# Autodesk Inventor assembly: ProvedoSenzor
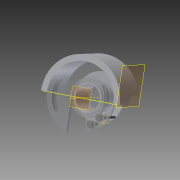
[picture p0: Inventor's stored thumbnail of the model, 180x180]
Saved by Autodesk Inventor 2015 (Build 190159000, 159)
## iProperties
Created: 2014-11-14
Part Number: ProvedoSenzor
Document SubType Name: Assembly
Designer: laca
Author: laca
## Documents named in this file (12)
- C:\Users\laca\Desktop\iRoobo2014Ver3\ProvedoSenzor.iam
- C:\Users\laca\Desktop\iRoobo2014Ver3\BurkolatPVCszenzor.ipt
- C:\Users\laca\Desktop\iRoobo2014Ver3\PorvedoRogzitesAVazhoz.ipt
- C:\Users\laca\Desktop\iRoobo2014Ver3\BurkolatPVCszenzorFedel.ipt
- C:\Users\laca\Desktop\iRoobo2014Ver3\SzenzorSzuportKerek.ipt
- C:\Users\laca\Desktop\iRoobo2014Ver3\InkrementalisOptikaiErzekelo.ipt
- C:\Users\laca\Desktop\iRoobo2014Ver3\InkrementalisFolia.ipt
- C:\Users\laca\Desktop\iRoobo2014Ver3\MerevitesInkrementalisFolia.ipt
- C:\Users\laca\Desktop\iRoobo2014Ver3\Alatet3csavarhoz.ipt
- C:\Users\laca\Desktop\iRoobo2014Ver3\Fi3es40mmcsavar Hexagon.ipt
- C:\Users\laca\Desktop\iRoobo2014Ver3\3asAnya.ipt
- C:\Users\laca\Desktop\iRoobo2014Ver3\KisLemezcsavar.ipt
## Components (22 placed, 11 different names)
1. PorvedoRogzitesAVazhoz:1 — Rotational:23, Insert:4, Flush:2, Rotational:28, Rotational:29, Rotational:32, Rotational:33
2. BurkolatPVCszenzorFedel:1
3. SzenzorSzuportKerek:1 — Rigid:1, Insert:2, Insert:3, Insert:4, Mate:1
4. InkrementalisFolia:1
5. MerevitesInkrementalisFolia:1 — Rigid:1, Rigid:3
6. MerevitesInkrementalisFolia:2 — Rigid:3
7. KisLemezcsavar:1 — Insert:2
8. KisLemezcsavar:2 — Insert:3
9. BurkolatPVCszenzor:2 — Rotational:23, Flush:2
10. InkrementalisOptikaiErzekelo:2 — Cylindrical:1, Rotational:26, Rotational:27, Rotational:34, Rotational:35, Cylindrical:2
11. 3asAnya:5 — Rotational:27
12. 3asAnya:4 — Rotational:26
13. 3asAnya:2 — Rotational:25
14. Alatet3csavarhoz:6 — Rotational:25, Rotational:29
15. Alatet3csavarhoz:7 — Rotational:28
16. Fi3es40mmcsavar Hexagon:3 — Cylindrical:1
17. Alatet3csavarhoz:8 — Rotational:33
18. 3asAnya:6
19. Alatet3csavarhoz:9 — Rotational:32
20. Fi3es40mmcsavar Hexagon:4 — Cylindrical:2
21. 3asAnya:7 — Rotational:35
22. 3asAnya:8 — Rotational:34
## Relationships (22: RevoluteJoint 13, Insert 3, WeldJoint 2, CylindricalJoint 2, Flush 1, Mate 1)
- Rigid:1 [WeldJoint] (-8 mm): SzenzorSzuportKerek:1 ↔ MerevitesInkrementalisFolia:1
- [RevoluteJoint]: Alatet3csavarhoz:7 ↔ Fi3es40mmcsavar Hexagon:3
- Insert:2: SzenzorSzuportKerek:1 ↔ KisLemezcsavar:1
- Insert:3: SzenzorSzuportKerek:1 ↔ KisLemezcsavar:2
- Rigid:3 [WeldJoint]: MerevitesInkrementalisFolia:1 ↔ MerevitesInkrementalisFolia:2
- Rotational:23 [RevoluteJoint]: PorvedoRogzitesAVazhoz:1 ↔ BurkolatPVCszenzor:2
- Insert:4: PorvedoRogzitesAVazhoz:1 ↔ SzenzorSzuportKerek:1
- Rotational:25 [RevoluteJoint]: 3asAnya:2 ↔ Alatet3csavarhoz:6
- Cylindrical:1: InkrementalisOptikaiErzekelo:2 ↔ Fi3es40mmcsavar Hexagon:3
- Rotational:26 [RevoluteJoint]: InkrementalisOptikaiErzekelo:2 ↔ 3asAnya:4
- Rotational:27 [RevoluteJoint]: InkrementalisOptikaiErzekelo:2 ↔ 3asAnya:5
- Flush:2: PorvedoRogzitesAVazhoz:1 ↔ BurkolatPVCszenzor:2
- Mate:1: SzenzorSzuportKerek:1
- Rotational:28 [RevoluteJoint]: PorvedoRogzitesAVazhoz:1 ↔ Alatet3csavarhoz:7
- Rotational:29 [RevoluteJoint]: PorvedoRogzitesAVazhoz:1 ↔ Alatet3csavarhoz:6
- [RevoluteJoint]: Alatet3csavarhoz:9 ↔ Fi3es40mmcsavar Hexagon:4
- [RevoluteJoint]: Alatet3csavarhoz:8 ↔ 3asAnya:6
- Rotational:32 [RevoluteJoint]: PorvedoRogzitesAVazhoz:1 ↔ Alatet3csavarhoz:9
- Rotational:33 [RevoluteJoint]: PorvedoRogzitesAVazhoz:1 ↔ Alatet3csavarhoz:8
- Rotational:34 [RevoluteJoint]: InkrementalisOptikaiErzekelo:2 ↔ 3asAnya:8
- Rotational:35 [RevoluteJoint]: InkrementalisOptikaiErzekelo:2 ↔ 3asAnya:7
- Cylindrical:2: InkrementalisOptikaiErzekelo:2 ↔ Fi3es40mmcsavar Hexagon:4
## Named parameters: d72_d43 = 0 mm, d73_d46 = -40.344676 deg, d149_d123 = 0 mm, d150_d124 = 3.571609 deg, d151_d72_d43 = 0 mm, d152_d73_d46 = 97.618508 deg
